# Autodesk Inventor assembly: Chain Drive2_MIR
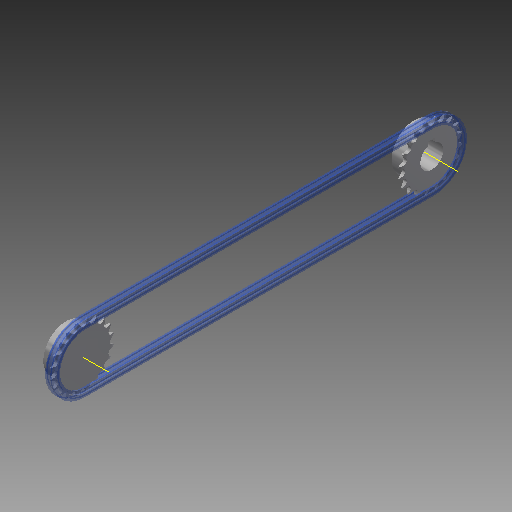
[picture p0: Inventor's stored thumbnail of the model, 512x512]
Saved by Autodesk Inventor 2019.4 (Build 234330000, 330)
## iProperties
Created: 2019-12-14
Part Number: Chain Drive2_MIR
Document SubType Name: Assembly
Designer: Mark
Mass: 317.317 g
Surface Area: 397.389 cm^2
Volume: 68.819 cm^3
Density: 4.61089 g/cm^3
Author: admin
## Documents named in this file (4)
- C:\Users\Mark\Desktop\7738 Helion Engineering\7738-CAD-prep\Offline CAD\WCD Mk3\Design Accelerator\Chain Drive2_MIR.iam
- C:\Users\Mark\Desktop\7738 Helion Engineering\7738-CAD-prep\Offline CAD\WCD Mk3\Design Accelerator\Roller Chain2_MIR.ipt
- C:\Users\Mark\Desktop\7738 Helion Engineering\7738-CAD-prep\Offline CAD\WCD Mk3\Design Accelerator\Roller Chain Sprocket12_MIR.ipt
- C:\Users\Mark\Desktop\7738 Helion Engineering\7738-CAD-prep\Offline CAD\WCD Mk3\Design Accelerator\Roller Chain Sprocket22_MIR.ipt
## Components (3 placed, 3 different names)
1. Roller Chain2_MIR:1 — Mate:2, Mate:1, Flush:1, Mate:4, Mate:3, Flush:2
2. Roller Chain Sprocket12_MIR:1 — Mate:2, Mate:1, Flush:1, Rotation:1
3. Roller Chain Sprocket22_MIR:1 — Mate:4, Mate:3, Flush:2, Rotation:1
## Relationships (7: Mate 4, Flush 2, RelateRotation 1)
- Mate:2: Roller Chain2_MIR:1 ↔ Roller Chain Sprocket12_MIR:1
- Mate:1: Roller Chain2_MIR:1 ↔ Roller Chain Sprocket12_MIR:1
- Flush:1: Roller Chain2_MIR:1 ↔ Roller Chain Sprocket12_MIR:1
- Mate:4: Roller Chain2_MIR:1 ↔ Roller Chain Sprocket22_MIR:1
- Mate:3: Roller Chain2_MIR:1 ↔ Roller Chain Sprocket22_MIR:1
- Flush:2: Roller Chain2_MIR:1 ↔ Roller Chain Sprocket22_MIR:1
- Rotation:1 [RelateRotation] (1 ul): Roller Chain Sprocket12_MIR:1 ↔ Roller Chain Sprocket22_MIR:1
